# Autodesk Inventor assembly: 2x8
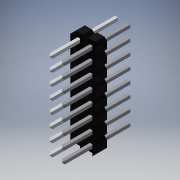
[picture p0: Inventor's stored thumbnail of the model, 180x180]
Saved by Autodesk Inventor 2019 (Build 230136000, 136)
## iProperties
Created: 2019-06-02
Part Number: 2x8
Document SubType Name: Assembly
Designer: jg_ma
Author: jg_ma
## Documents named in this file (2)
- D:\Desktop\Eletronica_Mecanica\MainBoard_V1.1\Pinos\2x8.iam
- D:\Desktop\Eletronica_Mecanica\MainBoard_V1.1\Pinos\Pino_180(2).ipt
## Components (8 placed, 1 different names)
1. Pino_180(2):1 — Mate:1, Flush:7, Flush:15
2. Pino_180(2):2 — Mate:1, Mate:2, Flush:6, Flush:7, Flush:14, Flush:15
3. Pino_180(2):3 — Mate:2, Mate:3, Flush:5, Flush:6, Flush:13, Flush:14
4. Pino_180(2):4 — Mate:3, Mate:4, Flush:4, Flush:5, Flush:12, Flush:13
5. Pino_180(2):5 — Mate:7, Flush:1, Flush:9
6. Pino_180(2):6 — Mate:6, Mate:7, Flush:1, Flush:2, Flush:9, Flush:10
7. Pino_180(2):7 — Mate:5, Mate:6, Flush:2, Flush:3, Flush:8, Flush:10, Flush:11
8. Pino_180(2):8 — Mate:4, Mate:5, Flush:3, Flush:4, Flush:8, Flush:11, Flush:12
## Relationships (22: Flush 15, Mate 7)
- Mate:1: Pino_180(2):1 ↔ Pino_180(2):2
- Mate:2: Pino_180(2):2 ↔ Pino_180(2):3
- Mate:3: Pino_180(2):3 ↔ Pino_180(2):4
- Mate:4: Pino_180(2):4 ↔ Pino_180(2):8
- Mate:5: Pino_180(2):7 ↔ Pino_180(2):8
- Mate:6: Pino_180(2):6 ↔ Pino_180(2):7
- Mate:7: Pino_180(2):5 ↔ Pino_180(2):6
- Flush:1: Pino_180(2):5 ↔ Pino_180(2):6
- Flush:2: Pino_180(2):6 ↔ Pino_180(2):7
- Flush:3: Pino_180(2):7 ↔ Pino_180(2):8
- Flush:4: Pino_180(2):4 ↔ Pino_180(2):8
- Flush:5: Pino_180(2):3 ↔ Pino_180(2):4
- Flush:6: Pino_180(2):2 ↔ Pino_180(2):3
- Flush:7: Pino_180(2):1 ↔ Pino_180(2):2
- Flush:8: Pino_180(2):7 ↔ Pino_180(2):8
- Flush:9: Pino_180(2):5 ↔ Pino_180(2):6
- Flush:10: Pino_180(2):6 ↔ Pino_180(2):7
- Flush:11: Pino_180(2):7 ↔ Pino_180(2):8
- Flush:12: Pino_180(2):4 ↔ Pino_180(2):8
- Flush:13: Pino_180(2):3 ↔ Pino_180(2):4
- Flush:14: Pino_180(2):2 ↔ Pino_180(2):3
- Flush:15: Pino_180(2):1 ↔ Pino_180(2):2
